# Autodesk Inventor assembly: Z Motor Assmbly_CPY
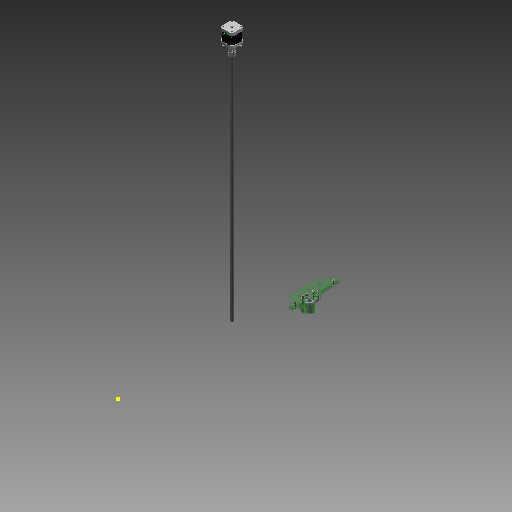
[picture p0: Inventor's stored thumbnail of the model, 512x512]
Saved by Autodesk Inventor 2017 (Build 210142000, 142)
## iProperties
Created: 2016-07-25
Part Number: Z Motor Assmbly_CPY
Document SubType Name: Assembly
Designer: User
Author: User
## Documents named in this file (7)
- C:\All INVENTOR\SL-Inventor\SL-Beast 3D Printer\Z Motor Assmbly_CPY.iam
- C:\All INVENTOR\SL-Inventor\SL-Beast 3D Printer\Lead Screw-A_CPY.ipt
- C:\All INVENTOR\SL-Inventor\SL-Beast 3D Printer\Nema17_CPY.ipt
- C:\All INVENTOR\SL-Inventor\SL-Beast 3D Printer\en-US\ANSI B18.3.1M(6)\ANSI B18.3.1M - M3x0.5 x 10(1).ipt
- C:\All INVENTOR\SL-Inventor\SL-Beast 3D Printer\Acople Flexible_CPY.ipt
- C:\All INVENTOR\SL-Inventor\SL-Beast 3D Printer\en-US\CNS 4480\CNS 4480 - M3 x 5.ipt
- C:\All INVENTOR\SL-Inventor\SL-Beast 3D Printer\Rear-Bed-Holder.iam
## Components (12 placed, 6 different names)
1. Lead Screw-A_CPY:1 — Mate:1
2. Rear-Bed-Holder:1 [sub-assembly]
3. Nema17_CPY:1 — Mate:2
4. Forged Socket Head Cap Screw - Metric M3x0.5 x 10:1
5. Forged Socket Head Cap Screw - Metric M3x0.5 x 10:2
6. Forged Socket Head Cap Screw - Metric M3x0.5 x 10:3
7. Forged Socket Head Cap Screw - Metric M3x0.5 x 10:4
8. Acople Flexible_CPY:1 — Mate:1, Mate:2, Mate:5, Mate:3, Mate:4
9. CNS 4480 M3 x 5:1 — Mate:5, Mate:3, Flush:1
10. CNS 4480 M3 x 5:2 — Flush:1, Mate:4
11. CNS 4480 M3 x 5:3
12. CNS 4480 M3 x 5:4
## Component patterns: (2 elements, first: CNS 4480 M3 x 5:1 + CNS 4480 M3 x 5:2)
## Relationships (6: Mate 5, Flush 1)
- Mate:1: Lead Screw-A_CPY:1 ↔ Acople Flexible_CPY:1
- Mate:2: Nema17_CPY:1 ↔ Acople Flexible_CPY:1
- Mate:5 (10 mm): Acople Flexible_CPY:1 ↔ CNS 4480 M3 x 5:1
- Mate:3: Acople Flexible_CPY:1 ↔ CNS 4480 M3 x 5:1
- Flush:1: CNS 4480 M3 x 5:1 ↔ CNS 4480 M3 x 5:2
- Mate:4: Acople Flexible_CPY:1 ↔ CNS 4480 M3 x 5:2
